# Autodesk Inventor assembly: RailVCoverCV_pointtestasm
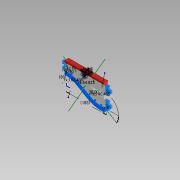
[picture p0: Inventor's stored thumbnail of the model, 180x180]
Saved by Autodesk Inventor 2021 (Build 250183000, 183)
## iProperties
Created: 2021-04-13
Part Number: RailVCoverCV_pointtestasm
Document SubType Name: Assembly
Designer: kumagai
Author: kumagai
## Documents named in this file (5)
- X:\Develop\CAD\PlaRails\Crossover\RailVCoverCV_pointtestasm.iam
- X:\Develop\CAD\PlaRails\Crossover\SingleCrossoverIA\SingleCrossover_PointA.iam
- X:\Develop\CAD\PlaRails\Crossover\SingleCrossoverIA.iam
- X:\Develop\CAD\PlaRails\Crossover\RailVCoverCV.ipt
- X:\Develop\CAD\PlaRails\Crossover\RailVCoverST.ipt
## Components (3 placed, 3 different names)
1. SingleCrossover_PointA:1 [sub-assembly] — メイト:1, メイト:2, メイト:3, メイト:4, メイト:5
2. RailVCoverCV:1 — メイト:1, メイト:2, メイト:3
3. RailVCoverST:1 — メイト:4, メイト:5
## Relationships (5: Mate 5)
- メイト:1 [Mate] (0.1 mm): SingleCrossover_PointA:1 ↔ RailVCoverCV:1
- メイト:2 [Mate]: SingleCrossover_PointA:1 ↔ RailVCoverCV:1
- メイト:3 [Mate]: SingleCrossover_PointA:1 ↔ RailVCoverCV:1
- メイト:4 [Mate]: SingleCrossover_PointA:1 ↔ RailVCoverST:1
- メイト:5 [Mate]: SingleCrossover_PointA:1 ↔ RailVCoverST:1
